# Autodesk Inventor assembly: AM14U3 Square Frame Half
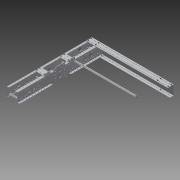
[picture p0: Inventor's stored thumbnail of the model, 180x180]
Saved by Autodesk Inventor 2018 (Build 220112000, 112)
## iProperties
Created: 2015-12-07
Part Number: AM14U3 Square Frame Half
Document SubType Name: Assembly
Designer: PhillipD
Author: PhillipD
Revision Number: ANY
## Documents named in this file (9)
- D:\FIRST 2018\FIRST 2018 Inventor\FIRST 2017 Drive Base\Parts\AM14U3 Square Frame Half.iam
- D:\FIRST 2018\FIRST 2018 Inventor\FIRST 2017 Drive Base\Parts\FHTS 0.25-20-0.75_FHTS 0.25-20-G-0.75-C.ipt
- D:\FIRST 2018\FIRST 2018 Inventor\FIRST 2017 Drive Base\Parts\Churro 3375.ipt
- D:\FIRST 2018\FIRST 2018 Inventor\FIRST 2017 Drive Base\Parts\Churro 20250.ipt
- D:\FIRST 2018\FIRST 2018 Inventor\FIRST 2017 Drive Base\Parts\AM14U3 End Sheet Square.ipt
- D:\FIRST 2018\FIRST 2018 Inventor\FIRST 2017 Drive Base\Parts\AM14U3 Inside Sheet Square.ipt
- D:\FIRST 2018\FIRST 2018 Inventor\FIRST 2017 Drive Base\Parts\AM14U3 Outside Sheet Square.ipt
- D:\FIRST 2018\FIRST 2018 Inventor\FIRST 2017 Drive Base\Parts\am-2954 AM14U2 2x3 Hole Bracket.ipt
- D:\FIRST 2018\FIRST 2018 Inventor\FIRST 2017 Drive Base\Parts\Nut_Screw.iam
## Components (38 placed, 21 different names)
1. FHTS 0.25-20-0.75_FHTS 0.25-20-G-0.75-C_98
2. FHTS 0.25-20-0.75_FHTS 0.25-20-G-0.75-C_99
3. FHTS 0.25-20-0.75_FHTS 0.25-20-G-0.75-C_100
4. FHTS 0.25-20-0.75_FHTS 0.25-20-G-0.75-C_101
5. FHTS 0.25-20-0.75_FHTS 0.25-20-G-0.75-C_102
6. FHTS 0.25-20-0.75_FHTS 0.25-20-G-0.75-C_103
7. FHTS 0.25-20-0.75_FHTS 0.25-20-G-0.75-C_104
8. FHTS 0.25-20-0.75_FHTS 0.25-20-G-0.75-C_105
9. FHTS 0.25-20-0.75_FHTS 0.25-20-G-0.75-C_106
10. FHTS 0.25-20-0.75_FHTS 0.25-20-G-0.75-C_107
11. Churro 3375_108
12. Churro 3375_109
13. Churro 3375_110
14. Churro 3375_111
15. Churro 20250_112
16. AM14U3 End Sheet Square_131 — Insert:14, Insert:15, Insert:16, Insert:17, Insert:18, Insert:20
17. AM14U3 Inside Sheet Square_132 — Insert:3, Insert:4, Insert:7, Insert:8, Insert:11, Insert:12
18. AM14U3 Outside Sheet Square_133 — Insert:1, Insert:2, Insert:5, Insert:6, Insert:9, Insert:10
19. am-2954 AM14U2 2x3 Hole Bracket_134
20. am-2954 AM14U2 2x3 Hole Bracket_135
21. Nut_Screw:1 [sub-assembly] — Insert:1
22. Nut_Screw:2 [sub-assembly] — Insert:4
23. Nut_Screw:3 [sub-assembly] — Insert:2
24. Nut_Screw:4 [sub-assembly] — Insert:3
25. Nut_Screw:5 [sub-assembly] — Insert:5
26. Nut_Screw:6 [sub-assembly] — Insert:8
27. Nut_Screw:7 [sub-assembly] — Insert:6
28. Nut_Screw:8 [sub-assembly] — Insert:7
29. Nut_Screw:9 [sub-assembly] — Insert:9
30. Nut_Screw:10 [sub-assembly] — Insert:10
31. Nut_Screw:11 [sub-assembly] — Insert:11
32. Nut_Screw:12 [sub-assembly] — Insert:12
33. Nut_Screw:13 [sub-assembly] — Insert:14
34. Nut_Screw:15 [sub-assembly] — Insert:16
35. Nut_Screw:16 [sub-assembly] — Insert:15
36. Nut_Screw:17 [sub-assembly] — Insert:17
37. Nut_Screw:18 [sub-assembly] — Insert:18
38. Nut_Screw:20 [sub-assembly] — Insert:20
## Relationships (18: Insert 18)
- Insert:1: AM14U3 Outside Sheet Square_133 ↔ Nut_Screw:1
- Insert:2: AM14U3 Outside Sheet Square_133 ↔ Nut_Screw:3
- Insert:3: AM14U3 Inside Sheet Square_132 ↔ Nut_Screw:4
- Insert:4: AM14U3 Inside Sheet Square_132 ↔ Nut_Screw:2
- Insert:5: AM14U3 Outside Sheet Square_133 ↔ Nut_Screw:5
- Insert:6: AM14U3 Outside Sheet Square_133 ↔ Nut_Screw:7
- Insert:7: AM14U3 Inside Sheet Square_132 ↔ Nut_Screw:8
- Insert:8: AM14U3 Inside Sheet Square_132 ↔ Nut_Screw:6
- Insert:9: AM14U3 Outside Sheet Square_133 ↔ Nut_Screw:9
- Insert:10: AM14U3 Outside Sheet Square_133 ↔ Nut_Screw:10
- Insert:11: AM14U3 Inside Sheet Square_132 ↔ Nut_Screw:11
- Insert:12: AM14U3 Inside Sheet Square_132 ↔ Nut_Screw:12
- Insert:14: AM14U3 End Sheet Square_131 ↔ Nut_Screw:13
- Insert:15: AM14U3 End Sheet Square_131 ↔ Nut_Screw:16
- Insert:16: AM14U3 End Sheet Square_131 ↔ Nut_Screw:15
- Insert:17: AM14U3 End Sheet Square_131 ↔ Nut_Screw:17
- Insert:18: AM14U3 End Sheet Square_131 ↔ Nut_Screw:18
- Insert:20: AM14U3 End Sheet Square_131 ↔ Nut_Screw:20
